# Autodesk Inventor assembly: lw_6_сборка_1
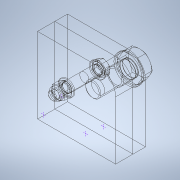
[picture p0: Inventor's stored thumbnail of the model, 180x180]
Saved by Autodesk Inventor 2021 (Build 250183000, 183)
## iProperties
Created: 2021-05-17
Part Number: lw_6_сборка_1
Document SubType Name: Assembly
Designer: davam
Author: davam
## Documents named in this file (8)
- C:\Users\davam\Desktop\лаб_6\lw_6_сборка_1.iam
- C:\Users\davam\Desktop\лаб_6\lw_6_part1.ipt
- C:\Users\davam\Desktop\лаб_6\lw_6_part2.ipt
- C:\Users\davam\Documents\Inventor\Content Center Files\R2021\ru-RU\ISO 7089\ISO 7089 - 20 - 140 HV(1).ipt
- C:\Users\davam\Documents\Inventor\Content Center Files\R2021\ru-RU\ISO 4017(1)\ISO 4017 - M20 x 110 - ISO.ipt
- C:\Users\davam\Documents\Inventor\Content Center Files\R2021\ru-RU\ISO 7041\ISO 7041 - M20 - ISO.ipt
- C:\Users\davam\Documents\Inventor\Content Center Files\R2021\ru-RU\Washer GOST 9065-75\Шайба 36 ГОСТ 9065-75.ipt
- C:\Users\davam\Documents\Inventor\Content Center Files\R2021\ru-RU\GOST ISO 4018\Винт с шестигранной головкой ГОСТ Р ISO 4018 - M36x90 - 4.6.ipt
## Components (8 placed, 7 different names)
1. lw_6_part1:1 — Заподлицо:1, Совмещение:1, Заподлицо:2, Совмещение:5
2. lw_6_part2:1 — Заподлицо:1, Совмещение:1, Заподлицо:2, Совмещение:2, Совмещение:3, Совмещение:4, Совмещение:6, Совмещение:7
3. ISO 7089 20:1 — Совмещение:2, Совмещение:3, Вставка:1
4. ISO 4017 M20 x 110:1 — Вставка:1
5. ISO 7089 20:2 — Совмещение:4, Совмещение:5, Вставка:2
6. ISO 7041 M20:1 — Вставка:2
7. Шайба ГОСТ 9065-75 36:1 — Совмещение:6, Совмещение:7, Вставка:3
8. ГОСТ ISO 4018 M36 x 90:1 — Вставка:3
## Relationships (12: Mate 7, Insert 3, Flush 2)
- Заподлицо:1 [Flush]: lw_6_part1:1 ↔ lw_6_part2:1
- Совмещение:1 [Mate]: lw_6_part1:1 ↔ lw_6_part2:1
- Заподлицо:2 [Flush]: lw_6_part1:1 ↔ lw_6_part2:1
- Совмещение:2 [Mate]: lw_6_part2:1 ↔ ISO 7089 20:1
- Совмещение:3 [Mate]: lw_6_part2:1 ↔ ISO 7089 20:1
- Вставка:1 [Insert]: ISO 7089 20:1 ↔ ISO 4017 M20 x 110:1
- Совмещение:4 [Mate]: lw_6_part2:1 ↔ ISO 7089 20:2
- Совмещение:5 [Mate]: lw_6_part1:1 ↔ ISO 7089 20:2
- Вставка:2 [Insert]: ISO 7089 20:2 ↔ ISO 7041 M20:1
- Совмещение:6 [Mate]: lw_6_part2:1 ↔ Шайба ГОСТ 9065-75 36:1
- Совмещение:7 [Mate]: lw_6_part2:1 ↔ Шайба ГОСТ 9065-75 36:1
- Вставка:3 [Insert]: Шайба ГОСТ 9065-75 36:1 ↔ ГОСТ ISO 4018 M36 x 90:1
